# Autodesk Inventor assembly: Ffoot2
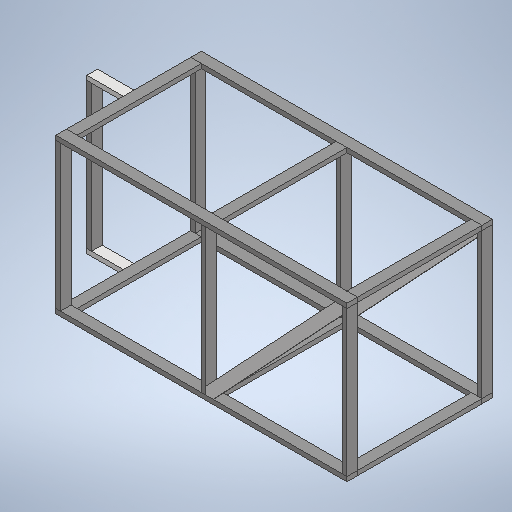
[picture p0: Inventor's stored thumbnail of the model, 512x512]
Saved by Autodesk Inventor 2026.1 (Build 301233000, 233)
## iProperties
Created: 2025-10-20
Part Number: Ffoot2
Document SubType Name: Assembly
Designer: jorda
Author: jorda
## Documents named in this file (6)
- C:\Users\jorda\OneDrive\Documents\GitHub\UofSC-ASME-Tiger-Burn-Design-2025\CAD\Legs\Front Foot\Ffoot2.iam
- C:\Users\jorda\OneDrive\Documents\GitHub\UofSC-ASME-Tiger-Burn-Design-2025\CAD\Legs\Back Foot\2x4x120.ipt
- C:\Users\jorda\OneDrive\Documents\GitHub\UofSC-ASME-Tiger-Burn-Design-2025\CAD\Legs\Back Foot\2x4x42.ipt
- C:\Users\jorda\OneDrive\Documents\GitHub\UofSC-ASME-Tiger-Burn-Design-2025\CAD\Legs\Back Foot\2x4x48.ipt
- C:\Users\jorda\OneDrive\Documents\GitHub\UofSC-ASME-Tiger-Burn-Design-2025\CAD\Legs\Front Foot\S_2x4x65.795.ipt
- C:\Users\jorda\OneDrive\Documents\GitHub\UofSC-ASME-Tiger-Burn-Design-2025\CAD\Head\2x4x12.ipt
## Components (21 placed, 5 different names)
1. 2x4x120:3 — Mate:1, Mate:2, Flush:1, Mate:5, Mate:25, Mate:26, Mate:29, Mate:30, Mate:33, Mate:53
2. 2x4x120:4 — Mate:3, Mate:4, Mate:6, Mate:27, Mate:28, Mate:31, Mate:32, Mate:37, Mate:46, Mate:48
3. 2x4x42:1 — Mate:1, Mate:2, Flush:1, Mate:3, Mate:4, Mate:52
4. 2x4x42:2 — Mate:5, Mate:6, Mate:38
5. 2x4x120:5 — Mate:21, Mate:22, Mate:23, Mate:24, Mate:35, Mate:51
6. 2x4x120:6 — Mate:39, Mate:41, Mate:42, Mate:43
7. 2x4x42:3 — Mate:21, Mate:22, Mate:36, Mate:43
8. 2x4x42:4 — Mate:23, Mate:24, Mate:50
9. 2x4x48:5 — Mate:25, Mate:26, Mate:34, Mate:41, Mate:42
10. 2x4x48:6 — Mate:27, Mate:28, Mate:47, Mate:49
11. 2x4x48:7 — Mate:29, Mate:30
12. 2x4x48:8 — Mate:31, Mate:32
13. 2x4x48:9 — Mate:33, Mate:34, Mate:40
14. 2x4x42:5 — Mate:35, Mate:36
15. 2x4x42:6 — Mate:37, Mate:38
16. S_2x4x65.795:1 — Mate:39, Mate:40
17. S_2x4x65.795:2 — Mate:46, Mate:47
18. 2x4x48:10 — Mate:48, Mate:49
19. 2x4x12:1 — Mate:50, Mate:51, Mate:54, Mate:55
20. 2x4x12:2 — Mate:52, Mate:53, Mate:56, Mate:57
21. 2x4x48:11 — Mate:54, Mate:55, Mate:56, Mate:57
## Relationships (42: Mate 41, Flush 1)
- Mate:1: 2x4x120:3 ↔ 2x4x42:1
- Mate:2: 2x4x120:3 ↔ 2x4x42:1
- Flush:1: 2x4x120:3 ↔ 2x4x42:1
- Mate:3: 2x4x120:4 ↔ 2x4x42:1
- Mate:4: 2x4x120:4 ↔ 2x4x42:1
- Mate:5: 2x4x120:3 ↔ 2x4x42:2
- Mate:6: 2x4x120:4 ↔ 2x4x42:2
- Mate:21: 2x4x120:5 ↔ 2x4x42:3
- Mate:22: 2x4x120:5 ↔ 2x4x42:3
- Mate:23: 2x4x120:5 ↔ 2x4x42:4
- Mate:24: 2x4x120:5 ↔ 2x4x42:4
- Mate:25: 2x4x120:3 ↔ 2x4x48:5
- Mate:26: 2x4x120:3 ↔ 2x4x48:5
- Mate:27: 2x4x120:4 ↔ 2x4x48:6
- Mate:28: 2x4x120:4 ↔ 2x4x48:6
- Mate:29: 2x4x120:3 ↔ 2x4x48:7
- Mate:30: 2x4x120:3 ↔ 2x4x48:7
- Mate:31: 2x4x120:4 ↔ 2x4x48:8
- Mate:32: 2x4x120:4 ↔ 2x4x48:8
- Mate:33: 2x4x120:3 ↔ 2x4x48:9
- Mate:34 (1219.2 mm): 2x4x48:5 ↔ 2x4x48:9
- Mate:35: 2x4x120:5 ↔ 2x4x42:5
- Mate:36 (1219.2 mm): 2x4x42:3 ↔ 2x4x42:5
- Mate:37: 2x4x120:4 ↔ 2x4x42:6
- Mate:38 (1219.2 mm): 2x4x42:2 ↔ 2x4x42:6
- Mate:39: 2x4x120:6 ↔ S_2x4x65.795:1
- Mate:40: 2x4x48:9 ↔ S_2x4x65.795:1
- Mate:41: 2x4x120:6 ↔ 2x4x48:5
- Mate:42: 2x4x120:6 ↔ 2x4x48:5
- Mate:43: 2x4x120:6 ↔ 2x4x42:3
- Mate:46: 2x4x120:4 ↔ S_2x4x65.795:2
- Mate:47: 2x4x48:6 ↔ S_2x4x65.795:2
- Mate:48: 2x4x120:4 ↔ 2x4x48:10
- Mate:49 (1219.2 mm): 2x4x48:6 ↔ 2x4x48:10
- Mate:50: 2x4x42:4 ↔ 2x4x12:1
- Mate:51 (565.15 mm): 2x4x120:5 ↔ 2x4x12:1
- Mate:52: 2x4x42:1 ↔ 2x4x12:2
- Mate:53 (565.15 mm): 2x4x120:3 ↔ 2x4x12:2
- Mate:54: 2x4x12:1 ↔ 2x4x48:11
- Mate:55: 2x4x12:1 ↔ 2x4x48:11
- Mate:56: 2x4x12:2 ↔ 2x4x48:11
- Mate:57: 2x4x12:2 ↔ 2x4x48:11
